# Autodesk Inventor assembly: certical cyinder asm
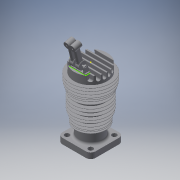
[picture p0: Inventor's stored thumbnail of the model, 180x180]
Saved by Autodesk Inventor 2018 (Build 220112000, 112)
## iProperties
Created: 2021-03-17
Part Number: certical cyinder asm
Document SubType Name: Assembly
Designer: Jyoti Soni
Author: Jyoti Soni
## Documents named in this file (4)
- C:\Users\Jyoti Soni\Desktop\asm\15032021\certical cyinder asm.iam
- C:\Users\Jyoti Soni\Desktop\asm\15032021\vertical cylinder.ipt
- C:\Users\Jyoti Soni\Desktop\asm\15032021\pin.ipt
- C:\Users\Jyoti Soni\Desktop\asm\15032021\knuckle.ipt
## Components (4 placed, 3 different names)
1. vertical cylinder:1 — Mate:1, Flush:1, Mate:3
2. pin:1 — Mate:1, Flush:1, Mate:2, Mate:4
3. knuckle:1 — Mate:2, Mate:3
4. knuckle:2 — Mate:4
## Relationships (5: Mate 4, Flush 1)
- Mate:1: vertical cylinder:1 ↔ pin:1
- Flush:1 (1 mm): vertical cylinder:1 ↔ pin:1
- Mate:2: pin:1 ↔ knuckle:1
- Mate:3 (2 mm): vertical cylinder:1 ↔ knuckle:1
- Mate:4: pin:1 ↔ knuckle:2
